# Autodesk Inventor assembly: FronPanelMilling
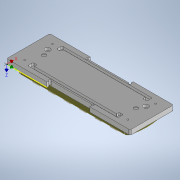
[picture p0: Inventor's stored thumbnail of the model, 180x180]
Saved by Autodesk Inventor 2022 (Build 260153000, 153)
## iProperties
Created: 2021-04-26
Part Number: FronPanelMilling
Document SubType Name: Assembly
Designer: lgnds
Author: lgnds
## Documents named in this file (4)
- D:\Drive\Chalmers\Fortsatt arbete WR\Design files\GPS Base Station\Manufacturing\FronPanelMilling.iam
- D:\Drive\Chalmers\Fortsatt arbete WR\Design files\GPS Base Station\Front_Panel\Panel\1009799_3D_Front_WaveRunner.ipt
- D:\Drive\Chalmers\Fortsatt arbete WR\Design files\GPS Base Station\Front_Panel\Panel\1009799_3D.ipt
- D:\Drive\Chalmers\Fortsatt arbete WR\Design files\GPS Base Station\Manufacturing\PanelJig v2.ipt
## Components (3 placed, 3 different names)
1. 1009799_3D_Front_WaveRunner:1
2. 1009799_3D:1 — Rigid:1
3. PanelJig v2:1 — Rigid:1
## Relationships (1: WeldJoint 1)
- Rigid:1 [WeldJoint]: 1009799_3D:1 ↔ PanelJig v2:1
